# Autodesk Inventor assembly: Shock Absorber
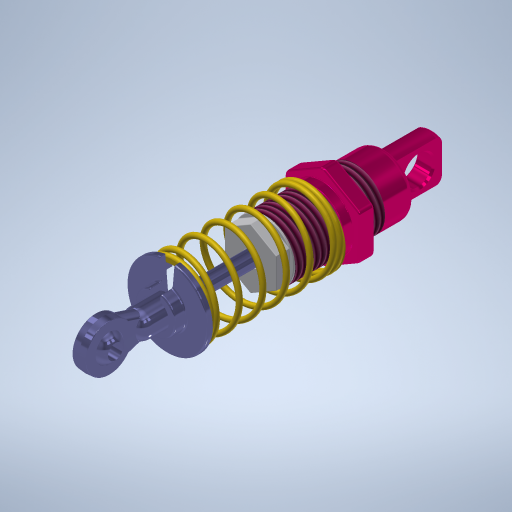
[picture p0: Inventor's stored thumbnail of the model, 512x512]
Saved by Autodesk Inventor 2023.1 (Build 271208000, 208)
## iProperties
Created: 2019-12-02
Part Number: Shock Absorber
Document SubType Name: Assembly
Designer: Jopa
Author: Jopa
## Documents named in this file (5)
- C:\Users\Arzum Naz Doğaner\OneDrive\Masaüstü\HUDSON süspansiyon\Shock Absorber.iam
- C:\Users\Arzum Naz Doğaner\OneDrive\Masaüstü\HUDSON süspansiyon\Shock Spring Adjustment Nut.ipt
- C:\Users\Arzum Naz Doğaner\OneDrive\Masaüstü\HUDSON süspansiyon\Suspension Spring.ipt
- C:\Users\Arzum Naz Doğaner\OneDrive\Masaüstü\HUDSON süspansiyon\Shock Body.iam
- C:\Users\Arzum Naz Doğaner\OneDrive\Masaüstü\HUDSON süspansiyon\Shock Strut.iam
## Components (4 placed, 4 different names)
1. Shock Spring Adjustment Nut:1 — Mate:1, Mate:2, Flush:1, Angle:1, Mate MID
2. Suspension Spring:1 — Mate:1, Mate:4, Mate MID
3. Shock Body:1 [sub-assembly] — Mate:2, Flush:1, Angle:1, Mate:3, Angle:2, Mate OPEN, Mate CLOSE
4. Shock Strut:1 [sub-assembly] — Mate:3, Mate:4, Angle:2, Mate OPEN, Mate CLOSE
## Relationships (10: Mate 7, Angle 2, Flush 1)
- Mate:1: Shock Spring Adjustment Nut:1 ↔ Suspension Spring:1
- Mate:2: Shock Spring Adjustment Nut:1 ↔ Shock Body:1
- Flush:1 (-10.1676 mm): Shock Spring Adjustment Nut:1 ↔ Shock Body:1
- Angle:1 (0 deg): Shock Spring Adjustment Nut:1 ↔ Shock Body:1
- Mate:3: Shock Body:1 ↔ Shock Strut:1
- Mate:4: Suspension Spring:1 ↔ Shock Strut:1
- Angle:2 (0 deg): Shock Body:1 ↔ Shock Strut:1
- Mate OPEN: Shock Body:1 ↔ Shock Strut:1
- Mate CLOSE: Shock Body:1 ↔ Shock Strut:1
- Mate MID: Shock Spring Adjustment Nut:1 ↔ Suspension Spring:1
